# Autodesk Inventor assembly: bearingAssembly
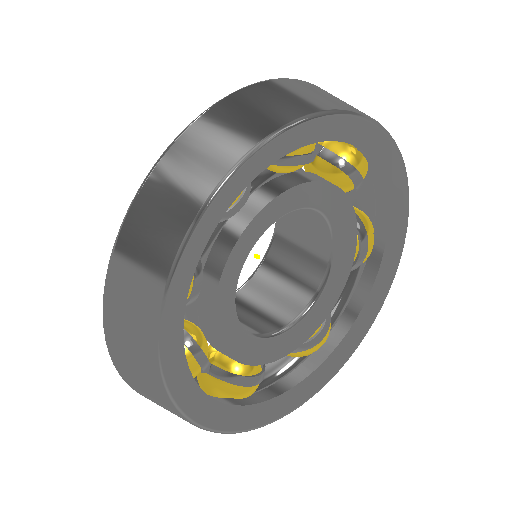
[picture p0: Inventor's stored thumbnail of the model, 512x512]
Saved by Autodesk Inventor 2025.2 (Build 292293000, 293)
## iProperties
Created: 2025-04-26
Part Number: bearingAssembly
Document SubType Name: Assembly
Designer: spars
Author: spars
## Documents named in this file (5)
- C:\Users\spars\OneDrive\Desktop\2nd Semester\Inventor\CAD@Start\bearingAssembly.iam
- C:\Users\spars\OneDrive\Desktop\2nd Semester\Inventor\bearing\outerring.ipt
- C:\Users\spars\OneDrive\Desktop\2nd Semester\Inventor\bearing\inner ring.ipt
- C:\Users\spars\OneDrive\Desktop\2nd Semester\Inventor\bearing\ball.ipt
- C:\Users\spars\OneDrive\Desktop\2nd Semester\Inventor\bearing\cage.ipt
## Components (12 placed, 4 different names)
1. outerring:1 — Mate:1, Mate:4, Flush:1
2. inner ring:1 — Mate:1, Mate:2, Tangent:1, Mate:3, Mate:4, Flush:1, Mate:5, Mate:6, Mate:7
3. cage:1 — Mate:5, Flush:2, Mate:8
4. cage:2 — Mate:6, Mate:7, Mate:8
5. ball:1 — Mate:2, Tangent:1, Mate:3, Flush:2, Angle:1
6. ball:2
7. ball:3
8. ball:4
9. ball:5
10. ball:6
11. ball:7
12. ball:8
## Component patterns: (8 elements, first: ball:1)
## Relationships (12: Mate 8, Flush 2, Tangent 1, Angle 1)
- Mate:1: outerring:1 ↔ inner ring:1
- Mate:2: inner ring:1 ↔ ball:1
- Tangent:1: inner ring:1 ↔ ball:1
- Mate:3: inner ring:1 ↔ ball:1
- Mate:4: outerring:1 ↔ inner ring:1
- Flush:1: outerring:1 ↔ inner ring:1
- Mate:5: inner ring:1 ↔ cage:1
- Flush:2: cage:1 ↔ ball:1
- Mate:6: inner ring:1 ↔ cage:2
- Mate:7: inner ring:1 ↔ cage:2
- Mate:8: cage:1 ↔ cage:2
- Angle:1 (0 deg): ball:1
